# Autodesk Inventor assembly: X_Slider
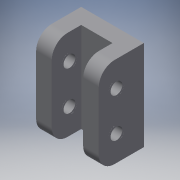
[picture p0: Inventor's stored thumbnail of the model, 180x180]
Saved by Autodesk Inventor 2019 (Build 230136000, 136)
## iProperties
Created: 2018-08-25
Part Number: X_Slider
Document SubType Name: Assembly
Designer: Julia
Author: Julia
## Documents named in this file (3)
- C:\Users\Julia\Documents\Inventor\3d_Drucker_v03_vertikaler_Gurt\X_Slider.iam
- C:\Users\Julia\Documents\Inventor\3d_Drucker_v03_vertikaler_Gurt\Metallstange_Slider.ipt
- C:\Users\Julia\Documents\Inventor\3d_Drucker_v03_vertikaler_Gurt\X_Slider_Part.ipt
## Components (5 placed, 2 different names)
1. Metallstange_Slider:1 — Mate:3, Flush:4
2. Metallstange_Slider:2 — Mate:1, Flush:1
3. Metallstange_Slider:3 — Mate:4, Flush:3
4. Metallstange_Slider:4 — Mate:2, Flush:2
5. X_Slider_Part:1 — Mate:1, Mate:2, Flush:1, Flush:2, Mate:3, Mate:4, Flush:3, Flush:4
## Relationships (8: Mate 4, Flush 4)
- Mate:1: Metallstange_Slider:2 ↔ X_Slider_Part:1
- Mate:2: Metallstange_Slider:4 ↔ X_Slider_Part:1
- Flush:1: Metallstange_Slider:2 ↔ X_Slider_Part:1
- Flush:2: Metallstange_Slider:4 ↔ X_Slider_Part:1
- Mate:3: Metallstange_Slider:1 ↔ X_Slider_Part:1
- Mate:4: Metallstange_Slider:3 ↔ X_Slider_Part:1
- Flush:3: Metallstange_Slider:3 ↔ X_Slider_Part:1
- Flush:4: Metallstange_Slider:1 ↔ X_Slider_Part:1
